# Autodesk Inventor assembly: MotorBoard_V1.0
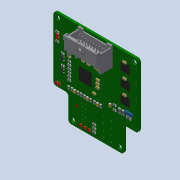
[picture p0: Inventor's stored thumbnail of the model, 180x180]
Saved by Autodesk Inventor 2020.4 (Build 244396000, 396)
## iProperties
Created: 2019-05-21
Part Number: MotorBoard_V1.0
Document SubType Name: Assembly
Designer: jg_ma
Sending System: Autodesk Translation Framework v8.2.0.1029
Preprocessor: ST-DEVELOPER v18
Title: c:\worker\convert-fusion-r04\tmp\job-1\22\output\files\b872785a-0138-4be1-bd62-03ee52a1c504\7be4d94e-0292-4e32-a0a1-3c0b01f39913.stp
## Documents named in this file (3)
- G:\Meu Drive\RobôCIn\Mecânica\SSL\2021\Inventor\first_floor\Components\MotorBoard\MOTORBOARD_V1.0.IAM
- G:\Meu Drive\RobôCIn\Mecânica\SSL\2021\Inventor\first_floor\Components\MotorBoard\PCB Component.iam
- G:\Meu Drive\RobôCIn\Mecânica\SSL\2021\Inventor\first_floor\Components\MotorBoard\559592030.ipt
## Components (2 placed, 2 different names)
1. PCB Component:1 [sub-assembly] — Mate:1, Flush:1
2. 559592030:1 — Mate:1, Flush:1
## Relationships (2: Mate 1, Flush 1)
- Mate:1: PCB Component:1 ↔ 559592030:1
- Flush:1: PCB Component:1 ↔ 559592030:1
